# Autodesk Inventor assembly: Assemlby_Scanner_v1
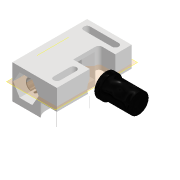
[picture p0: Inventor's stored thumbnail of the model, 180x180]
Saved by Autodesk Inventor 2022 (Build 260153000, 153)
## iProperties
Created: 2022-12-16
Part Number: Assemlby_Scanner_v1
Document SubType Name: Assembly
Designer: UC2
Author: UC2
## Documents named in this file (6)
- C:\Users\diederichbenedict\Dropbox\Dokumente\Promotion\PROJECTS\HoLiSheet\INVENTOR\Assemlby_Scanner_v1.iam
- C:\Users\diederichbenedict\Dropbox\Dokumente\Promotion\PROJECTS\HoLiSheet\INVENTOR\Assembly_Huawei_P30_Scanninglens.iam
- C:\Users\diederichbenedict\Dropbox\Dokumente\Promotion\PROJECTS\HoLiSheet\INVENTOR\30_Scanlens_Laseradaper_v1.ipt
- C:\Users\diederichbenedict\Dropbox\Dokumente\Promotion\PROJECTS\HoLiSheet\INVENTOR\00_CCTV_lens_M12_25mm_5mp.ipt
- C:\Users\diederichbenedict\Dropbox\Dokumente\Promotion\PROJECTS\HoLiSheet\INVENTOR\30_Scanlens_Laseradaper_lid_v1.ipt
- C:\Users\diederichbenedict\Dropbox\Dokumente\Promotion\PROJECTS\HoLiSheet\INVENTOR\00_Coverglass_50x24mm.ipt
## Components (6 placed, 5 different names)
1. Assembly_Huawei_P30_Scanninglens:1 [sub-assembly] — Fluchtend:1, Fluchtend:2, Fluchtend:3
2. 00_CCTV_lens_M12_25mm_5mp:1 — Passend:4
3. 30_Scanlens_Laseradaper_v1:1 — Fluchtend:1, Fluchtend:2, Fluchtend:3, Fluchtend:4, Fluchtend:5, Passend:2, Passend:3
4. 30_Scanlens_Laseradaper_lid_v1:1 — Fluchtend:4, Fluchtend:5, Winkel:1
5. 00_Coverglass_50x24mm:1 — Passend:2, Winkel:1, Passend:3, Passend:4, Fluchtend:6, Passend:5, Passend:6
6. 00_Coverglass_50x24mm:2 — Fluchtend:6, Passend:5, Passend:6
## Relationships (13: Flush 6, Mate 6, Angle 1)
- Fluchtend:1 [Flush]: Assembly_Huawei_P30_Scanninglens:1 ↔ 30_Scanlens_Laseradaper_v1:1
- Fluchtend:2 [Flush]: Assembly_Huawei_P30_Scanninglens:1 ↔ 30_Scanlens_Laseradaper_v1:1
- Fluchtend:3 [Flush]: Assembly_Huawei_P30_Scanninglens:1 ↔ 30_Scanlens_Laseradaper_v1:1
- [Mate]: Assembly_Huawei_P30_Scanninglens:1 ↔ 00_CCTV_lens_M12_25mm_5mp:1
- Fluchtend:4 [Flush]: 30_Scanlens_Laseradaper_v1:1 ↔ 30_Scanlens_Laseradaper_lid_v1:1
- Fluchtend:5 [Flush]: 30_Scanlens_Laseradaper_v1:1 ↔ 30_Scanlens_Laseradaper_lid_v1:1
- Passend:2 [Mate] (6 mm): 30_Scanlens_Laseradaper_v1:1 ↔ 00_Coverglass_50x24mm:1
- Winkel:1 [Angle] (0 deg): 30_Scanlens_Laseradaper_lid_v1:1 ↔ 00_Coverglass_50x24mm:1
- Passend:3 [Mate]: 30_Scanlens_Laseradaper_v1:1 ↔ 00_Coverglass_50x24mm:1
- Passend:4 [Mate]: 00_CCTV_lens_M12_25mm_5mp:1 ↔ 00_Coverglass_50x24mm:1
- Fluchtend:6 [Flush]: 00_Coverglass_50x24mm:1 ↔ 00_Coverglass_50x24mm:2
- Passend:5 [Mate]: 00_Coverglass_50x24mm:1 ↔ 00_Coverglass_50x24mm:2
- Passend:6 [Mate] (0.5 mm): 00_Coverglass_50x24mm:1 ↔ 00_Coverglass_50x24mm:2
## Named parameters: d3_d2 = 0 mm
